# Autodesk Inventor assembly: 20X20lift
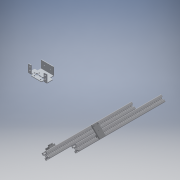
[picture p0: Inventor's stored thumbnail of the model, 180x180]
Saved by Autodesk Inventor 2017 (Build 210142000, 142)
## iProperties
Created: 2017-12-15
Part Number: 20X20lift
Document SubType Name: Assembly
Designer: User
Author: User
## Documents named in this file (5)
- C:\Robotics\CAD\2017-18_CAD\20X20lift.iam
- C:\Robotics\CAD\2017-18_CAD\Prototypes\Sliderfor2020.ipt
- C:\Robotics\CAD\COTSParts\Bosch Extrusion\Bosch 20x20 11.ipt
- C:\Robotics\CAD\2017-18_CAD\Prototypes\ServosSlideforLift.ipt
- C:\Robotics\CAD\COTSParts\Tetrix\39060_txm-standard servo bracket.ipt
## Components (6 placed, 4 different names)
1. Sliderfor2020:2 — Mate:10, Mate:11
2. Sliderfor2020:3 — Mate:5, Mate:6, Mate:8, Mate:9
3. Bosch 20x20 11:1 — Mate:5, Mate:6, Mate:11
4. Bosch 20x20 11:2 — Mate:8, Mate:9, Mate:10, Mate:12, Mate:13
5. ServosSlideforLift:1 — Mate:12, Mate:13
6. 39060_txm-standard servo bracket:1
## Relationships (8: Mate 8)
- Mate:5: Sliderfor2020:3 ↔ Bosch 20x20 11:1
- Mate:6: Sliderfor2020:3 ↔ Bosch 20x20 11:1
- Mate:8: Sliderfor2020:3 ↔ Bosch 20x20 11:2
- Mate:9: Sliderfor2020:3 ↔ Bosch 20x20 11:2
- Mate:10: Sliderfor2020:2 ↔ Bosch 20x20 11:2
- Mate:11: Sliderfor2020:2 ↔ Bosch 20x20 11:1
- Mate:12: Bosch 20x20 11:2 ↔ ServosSlideforLift:1
- Mate:13: Bosch 20x20 11:2 ↔ ServosSlideforLift:1
